# Autodesk Inventor assembly: 高さ調整用ミラー
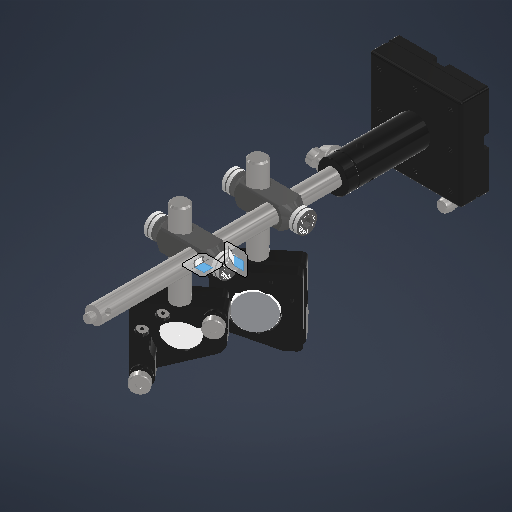
[picture p0: Inventor's stored thumbnail of the model, 512x512]
Saved by Autodesk Inventor 2026 (Build 300175050, 175E)
## iProperties
Created: 2025-07-11
Part Number: 高さ調整用ミラー
Document SubType Name: Assembly
Designer: jin20
Author: jin20
## Documents named in this file (6)
- C:\Users\jin20\Documents\装置CAD\RamanSystem\高さ調整用ミラー.iam
- C:\Users\jin20\Documents\装置CAD\RamanSystem\Stage\マグネットベース.ipt
- C:\Users\jin20\Documents\装置CAD\RamanSystem\Optics\ロッドスタンド.ipt
- C:\Users\jin20\Documents\装置CAD\RamanSystem\Optics\ロッド\ロッド_200mm.ipt
- C:\Users\jin20\Documents\装置CAD\RamanSystem\Optics\ロッドクランプ.ipt
- C:\Users\jin20\Documents\装置CAD\RamanSystem\Optics\ミラー.iam
## Components (7 placed, 5 different names)
1. マグネットベース:1 — 挿入:1
2. ロッドスタンド:1 — 挿入:1, リジッド:1
3. ロッド_200mm:1 — リジッド:1, 回転:3, 回転:4
4. ロッドクランプ:1 — 回転:3, 回転:5
5. ロッドクランプ:2 — 回転:4, 回転:6
6. ミラー:1 [sub-assembly] — 回転:5
7. ミラー:2 [sub-assembly] — 回転:6
## Relationships (6: RevoluteJoint 4, Insert 1, WeldJoint 1)
- 挿入:1 [Insert]: マグネットベース:1 ↔ ロッドスタンド:1
- リジッド:1 [WeldJoint] (-30 mm): ロッドスタンド:1 ↔ ロッド_200mm:1
- 回転:3 [RevoluteJoint] (-25 mm): ロッド_200mm:1 ↔ ロッドクランプ:1
- 回転:4 [RevoluteJoint] (15 mm): ロッド_200mm:1 ↔ ロッドクランプ:2
- 回転:5 [RevoluteJoint]: ロッドクランプ:1 ↔ ミラー:1
- 回転:6 [RevoluteJoint]: ロッドクランプ:2 ↔ ミラー:2
